# Autodesk Inventor assembly: 200-10-ROCKER-BEARING-ASM-01
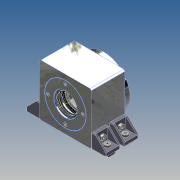
[picture p0: Inventor's stored thumbnail of the model, 180x180]
Saved by Autodesk Inventor 2018.2 (Build 222227000, 227)
## iProperties
Manager: feesmrt
Company: FRANCOR
Created: 2017-10-26
Part Number: 200-10-ROCKER-BEARING-ASM-01
Document SubType Name: Assembly
Designer: feesmrt
Mass: 1761.19 g
Surface Area: 1330.32 cm^2
Volume: 535.142 cm^3
Density: 3.29106 g/cm^3
Project: Rescue Robot
Cost Center: -
Description: Rocker Bearing
Engineer: feesmrt
Authority: feesmrt
Stock Number: 200-10-ROCKER-BEARING-ASM-01
Author: feesmrt
Title: Rocker Bearing
Subject: Rescue Robot
Revision Number: 1
## Documents named in this file (10)
- D:\Programmierung\FRANC0R\CAD\02-Rocker-Bogie-Robot\200-ROCKER-BOGIE\200-10-ROCKER-BEARING\200-10-ROCKER-BEARING-ASM-01.iam
- D:\Programmierung\FRANC0R\CAD\02-Rocker-Bogie-Robot\200-ROCKER-BOGIE\200-10-ROCKER-BEARING\200-10-ROCKER-BEARING-01.ipt
- D:\Programmierung\FRANC0R\CAD\02-Rocker-Bogie-Robot\900-COMPONENTS\900-20-BEARINGS\900-20-BEARINGS-3306-2RS-TN.ipt
- D:\Programmierung\FRANC0R\CAD\02-Rocker-Bogie-Robot\200-ROCKER-BOGIE\200-10-ROCKER-BEARING\200-10-ROCKER-BEARING-02.ipt
- D:\Programmierung\FRANC0R\CAD\02-Rocker-Bogie-Robot\900-COMPONENTS\900-30-SEALS\900-30-SEALS-DIN-3760-AS38x55x8-NBR.ipt
- D:\Programmierung\FRANC0R\CAD\02-Rocker-Bogie-Robot\200-ROCKER-BOGIE\200-10-ROCKER-BEARING\200-10-ROCKER-BEARING-03.ipt
- D:\Programmierung\FRANC0R\CAD\02-Rocker-Bogie-Robot\900-COMPONENTS\900-40-SCREWS\900-40-SCREWS-ISO10642_M3x8.ipt
- D:\Programmierung\FRANC0R\CAD\02-Rocker-Bogie-Robot\200-ROCKER-BOGIE\200-10-ROCKER-BEARING\200-10-ROCKER-BEARING-PROFILE-CONN-ASM-01.iam
- D:\Programmierung\FRANC0R\CAD\02-Rocker-Bogie-Robot\200-ROCKER-BOGIE\200-10-ROCKER-BEARING\200-10-ROCKER-BEARING-PROFILE-CONN-ASM-02.iam
- D:\Programmierung\FRANC0R\CAD\02-Rocker-Bogie-Robot\900-COMPONENTS\900-40-SCREWS\900-40-SCREWS-DIN7984_M5x12.ipt
## Components (19 placed, 9 different names)
1. 200-10-ROCKER-BEARING-01:1 — Passend:1, Passend:2, Passend:3, Passend:6, Passend:7, Passend:8, Passend:9, Passend:10, Passend:11, Passend:14, Passend:18, Passend:20, Passend:22, Passend:24, Passend:28, Passend:29, Passend:30, Passend:31, Winkel:1, Winkel:2, Passend:32
2. 900-20-BEARINGS-3306-2RS-TN:1 — Passend:1, Passend:2, Passend:3, Passend:4
3. 200-10-ROCKER-BEARING-02:1 — Passend:4, Passend:6, Passend:32, Passend:33, Passend:34
4. 900-30-SEALS-DIN-3760-AS38x55x8-NBR:1 — Passend:7, Passend:8
5. 200-10-ROCKER-BEARING-03:1 — Passend:9, Passend:10, Passend:11, Fluchtend:1
6. 200-10-ROCKER-BEARING-PROFILE-CONN-ASM-01:1 [sub-assembly] — Passend:18, Passend:24
7. 200-10-ROCKER-BEARING-PROFILE-CONN-ASM-01:3 [sub-assembly] — Passend:20, Passend:22
8. 200-10-ROCKER-BEARING-PROFILE-CONN-ASM-02:1 [sub-assembly] — Passend:28, Passend:31, Winkel:1
9. 200-10-ROCKER-BEARING-PROFILE-CONN-ASM-02:2 [sub-assembly] — Passend:29, Passend:30, Winkel:2
10. 900-40-SCREWS-ISO10642_M3x8:1 — Fluchtend:1, Passend:14
11. 900-40-SCREWS-ISO10642_M3x8:2
12. 900-40-SCREWS-ISO10642_M3x8:3
13. 900-40-SCREWS-ISO10642_M3x8:4
14. 900-40-SCREWS-DIN7984_M5x12:1 — Passend:33, Passend:34
15. 900-40-SCREWS-DIN7984_M5x12:2
16. 900-40-SCREWS-DIN7984_M5x12:3
17. 900-40-SCREWS-DIN7984_M5x12:4
18. 900-40-SCREWS-DIN7984_M5x12:5
19. 900-40-SCREWS-DIN7984_M5x12:6
## Component patterns: ISO10642_M3x8 (4 elements), DIN7984_M5x12 (6 elements)
## Relationships (25: Mate 22, Angle 2, Flush 1)
- Passend:1 [Mate]: 200-10-ROCKER-BEARING-01:1 ↔ 900-20-BEARINGS-3306-2RS-TN:1
- Passend:2 [Mate]: 200-10-ROCKER-BEARING-01:1 ↔ 900-20-BEARINGS-3306-2RS-TN:1
- Passend:3 [Mate]: 200-10-ROCKER-BEARING-01:1 ↔ 900-20-BEARINGS-3306-2RS-TN:1
- Passend:4 [Mate]: 900-20-BEARINGS-3306-2RS-TN:1 ↔ 200-10-ROCKER-BEARING-02:1
- Passend:6 [Mate]: 200-10-ROCKER-BEARING-01:1 ↔ 200-10-ROCKER-BEARING-02:1
- Passend:7 [Mate]: 200-10-ROCKER-BEARING-01:1 ↔ 900-30-SEALS-DIN-3760-AS38x55x8-NBR:1
- Passend:8 [Mate]: 200-10-ROCKER-BEARING-01:1 ↔ 900-30-SEALS-DIN-3760-AS38x55x8-NBR:1
- Passend:9 [Mate]: 200-10-ROCKER-BEARING-01:1 ↔ 200-10-ROCKER-BEARING-03:1
- Passend:10 [Mate]: 200-10-ROCKER-BEARING-01:1 ↔ 200-10-ROCKER-BEARING-03:1
- Passend:11 [Mate]: 200-10-ROCKER-BEARING-01:1 ↔ 200-10-ROCKER-BEARING-03:1
- Fluchtend:1 [Flush]: 200-10-ROCKER-BEARING-03:1 ↔ 900-40-SCREWS-ISO10642_M3x8:1
- Passend:14 [Mate]: 200-10-ROCKER-BEARING-01:1 ↔ 900-40-SCREWS-ISO10642_M3x8:1
- Passend:18 [Mate]: 200-10-ROCKER-BEARING-01:1 ↔ 200-10-ROCKER-BEARING-PROFILE-CONN-ASM-01:1
- Passend:20 [Mate]: 200-10-ROCKER-BEARING-01:1 ↔ 200-10-ROCKER-BEARING-PROFILE-CONN-ASM-01:3
- Passend:22 [Mate]: 200-10-ROCKER-BEARING-01:1 ↔ 200-10-ROCKER-BEARING-PROFILE-CONN-ASM-01:3
- Passend:24 [Mate]: 200-10-ROCKER-BEARING-01:1 ↔ 200-10-ROCKER-BEARING-PROFILE-CONN-ASM-01:1
- Passend:28 [Mate]: 200-10-ROCKER-BEARING-01:1 ↔ 200-10-ROCKER-BEARING-PROFILE-CONN-ASM-02:1
- Passend:29 [Mate]: 200-10-ROCKER-BEARING-01:1 ↔ 200-10-ROCKER-BEARING-PROFILE-CONN-ASM-02:2
- Passend:30 [Mate]: 200-10-ROCKER-BEARING-01:1 ↔ 200-10-ROCKER-BEARING-PROFILE-CONN-ASM-02:2
- Passend:31 [Mate]: 200-10-ROCKER-BEARING-01:1 ↔ 200-10-ROCKER-BEARING-PROFILE-CONN-ASM-02:1
- Winkel:1 [Angle] (0 deg): 200-10-ROCKER-BEARING-01:1 ↔ 200-10-ROCKER-BEARING-PROFILE-CONN-ASM-02:1
- Winkel:2 [Angle] (0 deg): 200-10-ROCKER-BEARING-01:1 ↔ 200-10-ROCKER-BEARING-PROFILE-CONN-ASM-02:2
- Passend:32 [Mate]: 200-10-ROCKER-BEARING-01:1 ↔ 200-10-ROCKER-BEARING-02:1
- Passend:33 [Mate]: 200-10-ROCKER-BEARING-02:1 ↔ 900-40-SCREWS-DIN7984_M5x12:1
- Passend:34 [Mate]: 200-10-ROCKER-BEARING-02:1 ↔ 900-40-SCREWS-DIN7984_M5x12:1
